# Autodesk Inventor assembly: XYZ
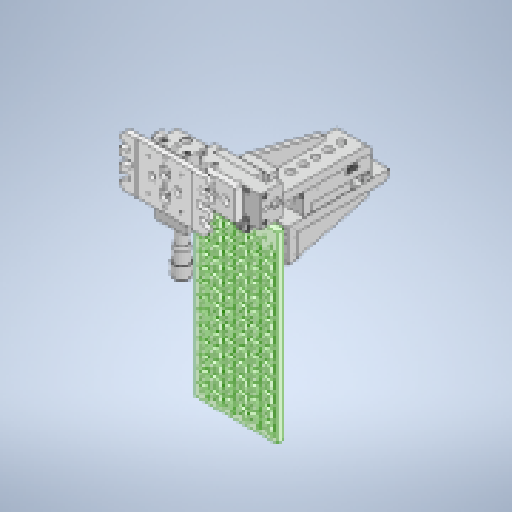
[picture p0: Inventor's stored thumbnail of the model, 512x512]
Saved by Autodesk Inventor 2026.1 (Build 301233000, 233)
## iProperties
Created: 2020-08-26
Part Number: XYZ
Document SubType Name: Assembly
Designer: Julian
Author: Julian
## Documents named in this file (6)
- C:\Users\user\Desktop\setup for publishing\XYZ.iam
- C:\Users\user\Desktop\setup for publishing\3UBP-04.ipt
- C:\Users\user\Desktop\setup for publishing\7T173-10.ipt
- C:\Users\user\Desktop\setup for publishing\2CP173-20.ipt
- C:\Users\user\Desktop\setup for publishing\2AB173-20.ipt
- C:\Users\user\Desktop\setup for publishing\Halterungsplatte.ipt
## Components (8 placed, 5 different names)
1. 3UBP-04:1 — Mate:1, Mate:2, Mate:3
2. 7T173-10:1 — Mate:1, Mate:2, Mate:3, Mate:6, Mate:28, Mate:29
3. 2CP173-20:1 — Mate:6, Mate:7, Mate:8, Mate:9, Mate:28, Mate:29
4. 7T173-10:2 — Mate:7, Mate:8, Mate:9, Mate:12, Mate:21, Mate:22
5. 2AB173-20:1 — Mate:12, Mate:13, Mate:14, Mate:15, Mate:21, Mate:22
6. 7T173-10:3 — Mate:13, Mate:14, Mate:15, Mate:18, Mate:23, Mate:24
7. 2AB173-20:2 — Mate:18, Mate:23, Mate:24, Mate:31, Mate:32, Passend:30
8. Halterungsplatte:1 — Passend:30, Mate:31, Mate:32
## Relationships (21: Mate 21)
- Mate:1: 3UBP-04:1 ↔ 7T173-10:1
- Mate:2: 3UBP-04:1 ↔ 7T173-10:1
- Mate:3: 3UBP-04:1 ↔ 7T173-10:1
- Mate:6: 7T173-10:1 ↔ 2CP173-20:1
- Mate:7: 2CP173-20:1 ↔ 7T173-10:2
- Mate:8: 2CP173-20:1 ↔ 7T173-10:2
- Mate:9: 2CP173-20:1 ↔ 7T173-10:2
- Mate:12: 7T173-10:2 ↔ 2AB173-20:1
- Mate:13: 2AB173-20:1 ↔ 7T173-10:3
- Mate:14: 2AB173-20:1 ↔ 7T173-10:3
- Mate:15: 2AB173-20:1 ↔ 7T173-10:3
- Mate:18: 7T173-10:3 ↔ 2AB173-20:2
- Mate:21: 7T173-10:2 ↔ 2AB173-20:1
- Mate:22: 7T173-10:2 ↔ 2AB173-20:1
- Mate:23: 7T173-10:3 ↔ 2AB173-20:2
- Mate:24: 7T173-10:3 ↔ 2AB173-20:2
- Mate:28: 7T173-10:1 ↔ 2CP173-20:1
- Mate:29 (0.5 mm): 7T173-10:1 ↔ 2CP173-20:1
- Passend:30 [Mate]: 2AB173-20:2 ↔ Halterungsplatte:1
- Mate:31: 2AB173-20:2 ↔ Halterungsplatte:1
- Mate:32: 2AB173-20:2 ↔ Halterungsplatte:1
